# Autodesk Inventor assembly: Ensamble Maquina GRAFCET
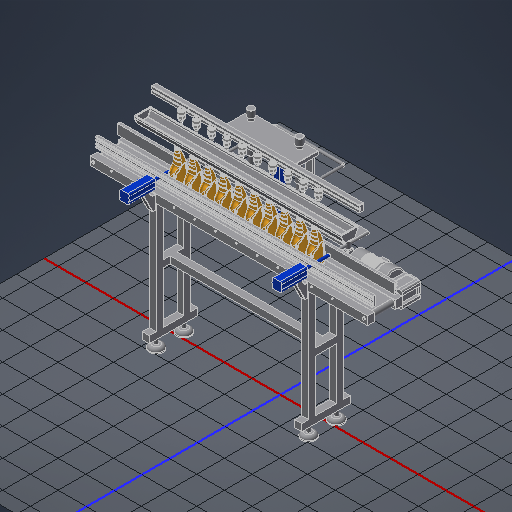
[picture p0: Inventor's stored thumbnail of the model, 512x512]
Saved by Autodesk Inventor 2026 (Build 300175000, 175)
## iProperties
Created: 2025-05-13
Part Number: Ensamble Maquina GRAFCET
Document SubType Name: Assembly
Designer: feder
Author: feder
## Documents named in this file (6)
- C:\Users\feder\OneDrive - Universidad de Antioquia\Desktop\UdeA\2025-1\Potencia\Trabajo GRAFCET\Maquina\Ensamble Maquina GRAFCET.iam
- C:\Users\feder\OneDrive - Universidad de Antioquia\Desktop\UdeA\2025-1\Potencia\Trabajo GRAFCET\Maquina\Banda Transporte.ipt
- C:\Users\feder\OneDrive - Universidad de Antioquia\Desktop\UdeA\2025-1\Potencia\Trabajo GRAFCET\Maquina\Soporte Boquillas.ipt
- C:\Users\feder\OneDrive - Universidad de Antioquia\Desktop\UdeA\2025-1\Potencia\Trabajo GRAFCET\Maquina\Boquilla.ipt
- C:\Users\feder\OneDrive - Universidad de Antioquia\Desktop\UdeA\2025-1\Potencia\Trabajo GRAFCET\Maquina\Botella Aceite.ipt
- C:\Users\feder\OneDrive - Universidad de Antioquia\Desktop\UdeA\2025-1\Potencia\Trabajo GRAFCET\Maquina\Bandeja Limpieza.ipt
## Components (23 placed, 5 different names)
1. Banda Transporte:1 — Mate:1, Mate:2, Mate:5, Tangent:1, Mate:6
2. Soporte Boquillas:1 — Mate:1, Mate:2, Mate:3, Mate:4, Flush:1, Mate:6
3. Bandeja Limpieza:1
4. Botella Aceite:1 — Mate:5, Tangent:1
5. Botella Aceite:2
6. Botella Aceite:3
7. Botella Aceite:4
8. Botella Aceite:5
9. Botella Aceite:6
10. Botella Aceite:7
11. Botella Aceite:8
12. Botella Aceite:9
13. Botella Aceite:10
14. Boquilla:1 — Mate:3, Mate:4, Flush:1
15. Boquilla:2
16. Boquilla:3
17. Boquilla:4
18. Boquilla:5
19. Boquilla:6
20. Boquilla:7
21. Boquilla:8
22. Boquilla:9
23. Boquilla:10
## Component patterns: (10 elements, first: Botella Aceite:1), (10 elements, first: Boquilla:1)
## Relationships (8: Mate 6, Tangent 1, Flush 1)
- Mate:1: Banda Transporte:1 ↔ Soporte Boquillas:1
- Mate:2: Banda Transporte:1 ↔ Soporte Boquillas:1
- Mate:3: Soporte Boquillas:1 ↔ Boquilla:1
- Mate:4: Soporte Boquillas:1 ↔ Boquilla:1
- Mate:5: Banda Transporte:1 ↔ Botella Aceite:1
- Tangent:1 (52 mm): Banda Transporte:1 ↔ Botella Aceite:1
- Flush:1 (226.467 mm): Soporte Boquillas:1 ↔ Boquilla:1
- Mate:6: Banda Transporte:1 ↔ Soporte Boquillas:1
